# Autodesk Inventor assembly: Application_Telescopes_v3
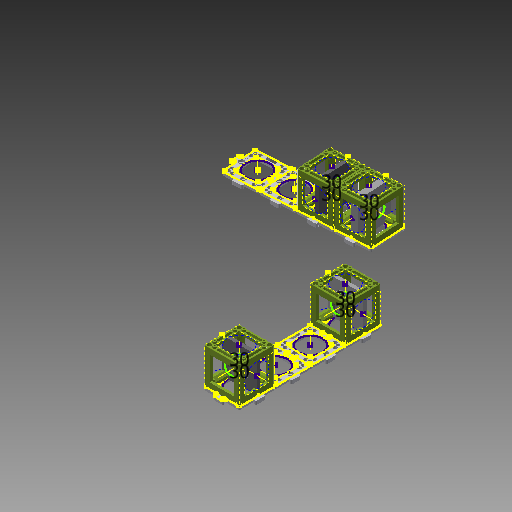
[picture p0: Inventor's stored thumbnail of the model, 512x512]
Saved by Autodesk Inventor 2019 (Build 230136000, 136)
## iProperties
Created: 2020-11-19
Part Number: Application_Telescopes_v3
Document SubType Name: Assembly
Designer: marsikovabarbora
Author: marsikovabarbora
## Documents named in this file (5)
- C:\Users\marsikovabarbora\Dropbox\UC2\02_CAD\INVENTOR\uc2_v3\Application_Telescopes_v3.iam
- C:\Users\marsikovabarbora\Dropbox\UC2\02_CAD\INVENTOR\uc2_v3\Assembly_base_4x1.iam
- C:\Users\marsikovabarbora\Dropbox\UC2\02_CAD\INVENTOR\uc2_v3\Assembly_Cube_Lens_holder_100mm_v3.iam
- C:\Users\marsikovabarbora\Dropbox\UC2\02_CAD\INVENTOR\uc2_v3\Assembly_Cube_Lens_holder_-50mm_v3.iam
- C:\Users\marsikovabarbora\Dropbox\UC2\02_CAD\INVENTOR\uc2_v3\Assembly_Cube_Lens_holder_50mm_v3.iam
## Components (6 placed, 4 different names)
1. Assembly_base_4x1:1 [sub-assembly] — Mate:1, Flush:1, Mate:4, Angle:2, Mate:5, Mate:6, Mate:7, Angle:3
2. Assembly_base_4x1:2 [sub-assembly] — Flush:1, Mate:2, Angle:1, Mate:3, Passend:8, Winkel:4, Passend:9
3. Assembly_Cube_Lens_holder_100mm_v3:1 [sub-assembly] — Mate:2, Angle:1, Mate:3
4. Assembly_Cube_Lens_holder_100mm_v3:2 [sub-assembly] — Mate:4, Angle:2, Mate:5
5. Assembly_Cube_Lens_holder_-50mm_v3:1 [sub-assembly] — Mate:6, Mate:7, Angle:3
6. Assembly_Cube_Lens_holder_50mm_v3:1 [sub-assembly] — Passend:8, Winkel:4, Passend:9
## Relationships (14: Mate 9, Angle 4, Flush 1)
- Mate:1: Assembly_base_4x1:1
- Flush:1: Assembly_base_4x1:1 ↔ Assembly_base_4x1:2
- Mate:2: Assembly_base_4x1:2 ↔ Assembly_Cube_Lens_holder_100mm_v3:1
- Angle:1 (0 deg): Assembly_base_4x1:2 ↔ Assembly_Cube_Lens_holder_100mm_v3:1
- Mate:3: Assembly_base_4x1:2 ↔ Assembly_Cube_Lens_holder_100mm_v3:1
- Mate:4: Assembly_base_4x1:1 ↔ Assembly_Cube_Lens_holder_100mm_v3:2
- Angle:2 (0 deg): Assembly_base_4x1:1 ↔ Assembly_Cube_Lens_holder_100mm_v3:2
- Mate:5: Assembly_base_4x1:1 ↔ Assembly_Cube_Lens_holder_100mm_v3:2
- Mate:6: Assembly_base_4x1:1 ↔ Assembly_Cube_Lens_holder_-50mm_v3:1
- Mate:7: Assembly_base_4x1:1 ↔ Assembly_Cube_Lens_holder_-50mm_v3:1
- Angle:3 (0 deg): Assembly_base_4x1:1 ↔ Assembly_Cube_Lens_holder_-50mm_v3:1
- Passend:8 [Mate]: Assembly_base_4x1:2 ↔ Assembly_Cube_Lens_holder_50mm_v3:1
- Winkel:4 [Angle] (0 deg): Assembly_base_4x1:2 ↔ Assembly_Cube_Lens_holder_50mm_v3:1
- Passend:9 [Mate]: Assembly_base_4x1:2 ↔ Assembly_Cube_Lens_holder_50mm_v3:1
